# Autodesk Inventor assembly: N_core
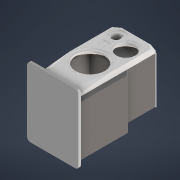
[picture p0: Inventor's stored thumbnail of the model, 180x180]
Saved by Autodesk Inventor 2022 (Build 260153070, 153G)
## iProperties
Created: 2021-11-16
Part Number: N_core
Document SubType Name: Assembly
Designer: kalugin_a
Mass: 21358.7 g
Surface Area: 28071.4 cm^2
Volume: 22490.4 cm^3
Density: 0.949678 g/cm^3
Author: kalugin_a
## Documents named in this file (18)
- C:\Users\kalugin_a\Documents\Inventor\TUTO\MELAS\Workspace\N_core.iam
- C:\Users\kalugin_a\Documents\Inventor\TUTO\MELAS\Workspace\N_Front.ipt
- C:\Users\kalugin_a\Documents\Inventor\TUTO\MELAS\Workspace\N_into_side.ipt
- C:\Users\kalugin_a\Documents\Inventor\TUTO\MELAS\Workspace\N-Back_into.ipt
- C:\Users\kalugin_a\Documents\Inventor\TUTO\MELAS\Workspace\N_Bottom.ipt
- C:\Users\kalugin_a\Documents\Inventor\TUTO\MELAS\Workspace\MID.ipt
- C:\Users\kalugin_a\Documents\Inventor\TUTO\MELAS\Workspace\N__side_sticker.ipt
- C:\Users\kalugin_a\Documents\Inventor\TUTO\MELAS\Workspace\N__side_sticker_MIR.ipt
- C:\Users\kalugin_a\Documents\Inventor\TUTO\MELAS\Workspace\WOOFER.ipt
- C:\Users\kalugin_a\Documents\Inventor\TUTO\MELAS\Workspace\MIDRange.ipt
- C:\Users\kalugin_a\Documents\Inventor\TUTO\MELAS\Workspace\Twitter.iam
- C:\Users\kalugin_a\Documents\Inventor\TUTO\MELAS\Workspace\TopCover.ipt
- C:\Users\kalugin_a\Documents\Inventor\TUTO\MELAS\Workspace\PowerSupply.ipt
- C:\Users\kalugin_a\Documents\Inventor\TUTO\MELAS\Workspace\midwall-0.ipt
- C:\Users\kalugin_a\Documents\Inventor\TUTO\MELAS\Workspace\FakeV.ipt
- C:\Users\kalugin_a\Documents\Inventor\TUTO\MELAS\Workspace\ArmDesk.ipt
- C:\Users\kalugin_a\Documents\Inventor\TUTO\MELAS\Workspace\PlateAMP.ipt
- C:\Users\kalugin_a\Documents\Inventor\TUTO\MELAS\Workspace\Stand_plate.ipt
## Components (19 placed, 18 different names)
1. N_Front:1 — Жесткий:17
2. N_into_side:1 — Жесткий:6, Заподлицо:1, Жесткий:11
3. N_into_side:2 — Жесткий:12, Жесткий:13, Жесткий:16
4. N-Back_into:1 — Жесткий:5
5. N_Flane_H — Жесткий:8, Жесткий:14
6. MID:1
7. N__side_sticker:1 — Жесткий:6
8. N__side_sticker_MIR:1 — Жесткий:5, Жесткий:16
9. N_Bottom:3 — Жесткий:9, Совмещение:1, Заподлицо:1, Жесткий:11, Жесткий:13, Жесткий:17
10. TopCover:1 — Жесткий:12
11. PowerSupply:1
12. midwall-0:1 — Жесткий:14
13. FakeV:1
14. ArmDesk:1 — Жесткий:8, Жесткий:9, Совмещение:1
15. PlateAMP:1
16. Stand_plate:1
17. Twitter:1 [sub-assembly]
18. MIDRange:1
19. WOOFER:2
## Relationships (12: WeldJoint 10, Mate 1, Flush 1)
- Жесткий:5 [WeldJoint]: N-Back_into:1 ↔ N__side_sticker_MIR:1
- Жесткий:6 [WeldJoint]: N_into_side:1 ↔ N__side_sticker:1
- Жесткий:8 [WeldJoint]: N_Flane_H ↔ ArmDesk:1
- Жесткий:9 [WeldJoint]: N_Bottom:3 ↔ ArmDesk:1
- Совмещение:1 [Mate]: N_Bottom:3 ↔ ArmDesk:1
- Заподлицо:1 [Flush]: N_into_side:1 ↔ N_Bottom:3
- Жесткий:11 [WeldJoint]: N_into_side:1 ↔ N_Bottom:3
- Жесткий:12 [WeldJoint]: N_into_side:2 ↔ TopCover:1
- Жесткий:13 [WeldJoint]: N_into_side:2 ↔ N_Bottom:3
- Жесткий:14 [WeldJoint] (-60 mm): N_Flane_H ↔ midwall-0:1
- Жесткий:16 [WeldJoint]: N_into_side:2 ↔ N__side_sticker_MIR:1
- Жесткий:17 [WeldJoint]: N_Front:1 ↔ N_Bottom:3
